# Autodesk Inventor assembly: 1103 ID Plate (with hardware)
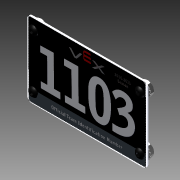
[picture p0: Inventor's stored thumbnail of the model, 180x180]
Saved by Autodesk Inventor 2012 (Build 160160000, 160)
## iProperties
Created: 2011-09-18
Part Number: 1103 ID Plate (with hardware)
Document SubType Name: Assembly
Designer: Wade
Author: Wade
## Documents named in this file (4)
- C:\Users\Wade\Documents\1103 Robot - CAD Assembly\1103 ID Plate (with hardware).iam
- C:\Users\Wade\Documents\24C VEX CAD Files\Screws & Nuts\Nut 8-32 Keps.ipt
- C:\Users\Wade\Documents\24C VEX CAD Files\Screws & Nuts\Screw 6-32 x 0.250''-Black.ipt
- C:\Users\Wade\Documents\1103 Robot - CAD Assembly\1103 ID Plate.ipt
## Components (9 placed, 3 different names)
1. Nut 8-32 Keps:1 — Mate:9, Mate:13
2. Screw 6-32 x 0.250''-Black:1 — Mate:1, Mate:5, Mate:10
3. Nut 8-32 Keps:2 — Mate:10, Mate:14
4. Screw 6-32 x 0.250''-Black:2 — Mate:4, Mate:11, Mate:18
5. Nut 8-32 Keps:3 — Mate:11, Mate:15
6. Screw 6-32 x 0.250''-Black:3 — Mate:3, Mate:9, Mate:17
7. Nut 8-32 Keps:4 — Mate:12, Mate:16
8. Screw 6-32 x 0.250''-Black:4 — Mate:2, Mate:6, Mate:12
9. 1103 ID Plate:1 — Mate:1, Mate:2, Mate:3, Mate:4, Mate:5, Mate:6, Mate:13, Mate:14, Mate:15, Mate:16, Mate:17, Mate:18
## Relationships (16: Mate 16)
- Mate:1: Screw 6-32 x 0.250''-Black:1 ↔ 1103 ID Plate:1
- Mate:2: Screw 6-32 x 0.250''-Black:4 ↔ 1103 ID Plate:1
- Mate:3: Screw 6-32 x 0.250''-Black:3 ↔ 1103 ID Plate:1
- Mate:4: Screw 6-32 x 0.250''-Black:2 ↔ 1103 ID Plate:1
- Mate:5 (0.254 mm): Screw 6-32 x 0.250''-Black:1 ↔ 1103 ID Plate:1
- Mate:6 (0.254 mm): Screw 6-32 x 0.250''-Black:4 ↔ 1103 ID Plate:1
- Mate:9: Nut 8-32 Keps:1 ↔ Screw 6-32 x 0.250''-Black:3
- Mate:10: Screw 6-32 x 0.250''-Black:1 ↔ Nut 8-32 Keps:2
- Mate:11: Screw 6-32 x 0.250''-Black:2 ↔ Nut 8-32 Keps:3
- Mate:12: Nut 8-32 Keps:4 ↔ Screw 6-32 x 0.250''-Black:4
- Mate:13 (1.1684 mm): Nut 8-32 Keps:1 ↔ 1103 ID Plate:1
- Mate:14 (1.1684 mm): Nut 8-32 Keps:2 ↔ 1103 ID Plate:1
- Mate:15 (1.1684 mm): Nut 8-32 Keps:3 ↔ 1103 ID Plate:1
- Mate:16 (1.1684 mm): Nut 8-32 Keps:4 ↔ 1103 ID Plate:1
- Mate:17 (0.254 mm): Screw 6-32 x 0.250''-Black:3 ↔ 1103 ID Plate:1
- Mate:18 (0.254 mm): Screw 6-32 x 0.250''-Black:2 ↔ 1103 ID Plate:1
